# Autodesk Inventor assembly: Robot
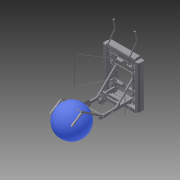
[picture p0: Inventor's stored thumbnail of the model, 180x180]
Saved by Autodesk Inventor 2013 (Build 170138000, 138)
## iProperties
Created: 2014-01-18
Part Number: Robot
Document SubType Name: Assembly
Designer: 272817
Author: 272817
## Documents named in this file (12)
- E:\Robotics\FRC\2014\CAD\Robot\Robot.iam
- E:\Robotics\FRC\2014\CAD\Robot\Frame\Robot Chassis 2014.iam
- E:\Robotics\FRC\2014\CAD\Robot\Bumpers\Bumpers.iam
- E:\Robotics\FRC\2014\CAD\Robot\Catapult\Arm\ArmSquare.iam
- E:\Robotics\FRC\2014\CAD\Robot\Catapult\Structure.iam
- E:\Robotics\FRC\2014\CAD\Robot\Ball.ipt
- E:\Robotics\FRC\2014\CAD\Robot\Catcher\CatchFrameLeft.ipt
- E:\Robotics\FRC\2014\CAD\Robot\Catcher\CatchFrameRight.ipt
- E:\Robotics\FRC\2014\CAD\Robot\Catcher\CatchStructure.iam
- E:\Robotics\FRC\2014\CAD\Robot\Pickup\Z-Plate-Gears.ipt
- E:\Robotics\FRC\2014\CAD\Robot\Pickup\Z-Arms-Gears.iam
- E:\Robotics\FRC\2014\CAD\Robot\Pickup\BumperStop.ipt
## Components (13 placed, 11 different names)
1. Robot Chassis 2014:1 [sub-assembly] — Mate:1, Mate:2, Mate:15, Mate:16, Mate:27, Angle:1, Mate:28, Mate:49, Mate:50, Mate:51, Mate:54, Mate:55
2. Bumpers:1 [sub-assembly] — Mate:1, Mate:2, Mate:17, Mate:35, Mate:49, Mate:59, Mate:61, Mate:62, Mate:63, Mate:64, Flush:1, Flush:2
3. ArmSquare:2 [sub-assembly] — Mate:18, Mate:19
4. Structure:1 [sub-assembly] — Mate:15, Mate:16, Mate:17, Mate:18, Mate:19
5. Z-Arms-Gears:1 [sub-assembly] — Mate:57, Mate:58, Mate:60
6. Z-Plate-Gears:1 — Mate:50, Mate:51, Mate:57, Mate:58, Mate:59
7. Z-Plate-Gears:2 — Mate:54, Mate:55, Mate:60
8. CatchStructure:1 [sub-assembly] — Mate:27, Angle:1, Mate:28, Mate:29, Mate:30, Mate:31, Mate:32, Mate:33, Mate:34
9. CatchFrameRight:1 — Mate:29, Mate:30, Mate:31
10. CatchFrameLeft:1 — Mate:32, Mate:33, Mate:34
11. Ball:1 — Mate:35
12. BumperStop:1 — Mate:61, Mate:62, Flush:1
13. BumperStop:2 — Mate:63, Mate:64, Flush:2
## Relationships (32: Mate 29, Flush 2, Angle 1)
- Mate:1: Robot Chassis 2014:1 ↔ Bumpers:1
- Mate:2 (0.127 mm): Robot Chassis 2014:1 ↔ Bumpers:1
- Mate:15: Robot Chassis 2014:1 ↔ Structure:1
- Mate:16: Robot Chassis 2014:1 ↔ Structure:1
- Mate:17 (50.8 mm): Bumpers:1 ↔ Structure:1
- Mate:18: ArmSquare:2 ↔ Structure:1
- Mate:19 (3.175 mm): ArmSquare:2 ↔ Structure:1
- Mate:27: Robot Chassis 2014:1 ↔ CatchStructure:1
- Angle:1 (0 deg): Robot Chassis 2014:1 ↔ CatchStructure:1
- Mate:28: Robot Chassis 2014:1 ↔ CatchStructure:1
- Mate:29 (6.35 mm): CatchStructure:1 ↔ CatchFrameRight:1
- Mate:30 (6.35 mm): CatchStructure:1 ↔ CatchFrameRight:1
- Mate:31: CatchStructure:1 ↔ CatchFrameRight:1
- Mate:32 (6.35 mm): CatchStructure:1 ↔ CatchFrameLeft:1
- Mate:33: CatchStructure:1 ↔ CatchFrameLeft:1
- Mate:34 (6.35 mm): CatchStructure:1 ↔ CatchFrameLeft:1
- Mate:35 (292.1 mm): Bumpers:1 ↔ Ball:1
- Mate:49 (-22.225 mm): Robot Chassis 2014:1 ↔ Bumpers:1
- Mate:50: Robot Chassis 2014:1 ↔ Z-Plate-Gears:1
- Mate:51: Robot Chassis 2014:1 ↔ Z-Plate-Gears:1
- Mate:54: Robot Chassis 2014:1 ↔ Z-Plate-Gears:2
- Mate:55: Robot Chassis 2014:1 ↔ Z-Plate-Gears:2
- Mate:57: Z-Arms-Gears:1 ↔ Z-Plate-Gears:1
- Mate:58: Z-Arms-Gears:1 ↔ Z-Plate-Gears:1
- Mate:59 (12.7 mm): Bumpers:1 ↔ Z-Plate-Gears:1
- Mate:60: Z-Arms-Gears:1 ↔ Z-Plate-Gears:2
- Mate:61: Bumpers:1 ↔ BumperStop:1
- Mate:62: Bumpers:1 ↔ BumperStop:1
- Mate:63: Bumpers:1 ↔ BumperStop:2
- Mate:64: Bumpers:1 ↔ BumperStop:2
- Flush:1 (-57.15 mm): Bumpers:1 ↔ BumperStop:1
- Flush:2 (57.15 mm): Bumpers:1 ↔ BumperStop:2
